# Autodesk Inventor assembly: inner
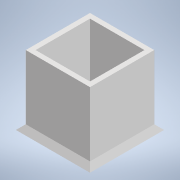
[picture p0: Inventor's stored thumbnail of the model, 180x180]
Saved by Autodesk Inventor 2021 (Build 250183000, 183)
## iProperties
Created: 2020-06-13
Part Number: inner
Document SubType Name: Assembly
Designer: Yatekii
Author: Yatekii
## Documents named in this file (3)
- C:\Users\Yatekii\repos\rcache\inner.iam
- C:\Users\Yatekii\repos\rcache\side.ipt
- C:\Users\Yatekii\repos\rcache\inner_side.ipt
## Components (5 placed, 2 different names)
1. side:1 — Mate:1, Mate:2
2. inner_side:1 — Rigid:2, Mate:1
3. inner_side:2 — Rigid:1, Rigid:2
4. inner_side:3 — Rigid:1, Rigid:3
5. inner_side:4 — Rigid:3, Mate:2
## Relationships (5: WeldJoint 3, Mate 2)
- Rigid:1 [WeldJoint]: inner_side:2 ↔ inner_side:3
- Rigid:2 [WeldJoint]: inner_side:1 ↔ inner_side:2
- Rigid:3 [WeldJoint]: inner_side:3 ↔ inner_side:4
- Mate:1: side:1 ↔ inner_side:1
- Mate:2: side:1 ↔ inner_side:4
